# Autodesk Inventor assembly: ANDGATEASSEMBLY
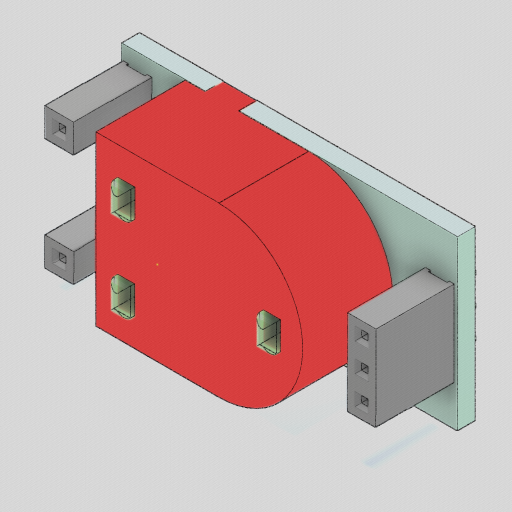
[picture p0: Inventor's stored thumbnail of the model, 512x512]
Saved by Autodesk Inventor 2024.3 (Build 283343000, 343)
## iProperties
Created: 2024-01-22
Part Number: ANDGATEASSEMBLY
Document SubType Name: Assembly
Designer: Jetsan
Author: Jetsan
## Documents named in this file (4)
- C:\Git\DigitalLogicProject\Models\ANDGATE\ANDGATEASSEMBLY.iam
- C:\Git\DigitalLogicProject\Models\LIGHTPIPING\LightPipe.ipt
- C:\Git\DigitalLogicProject\PCBS\GATE\GATE PCB.ipt
- C:\Git\DigitalLogicProject\Models\ANDGATE\ANDGATE.ipt
## Components (5 placed, 3 different names)
1. LightPipe:1 — Mate:3
2. LightPipe:2 — Mate:4
3. ANDGATE:1
4. GATE PCB:1 — Mate:3, Mate:4, Mate:10
5. LightPipe:3 — Mate:10
## Relationships (11: Mate 10, Flush 1)
- Mate:3: LightPipe:1 ↔ GATE PCB:1
- Mate:4: LightPipe:2 ↔ GATE PCB:1
- [Flush]: ANDGATE:1 ↔ GATE PCB:1
- [Mate]: ANDGATE:1 ↔ GATE PCB:1
- [Mate]: LightPipe:1 ↔ ANDGATE:1
- [Mate]: LightPipe:1 ↔ ANDGATE:1
- [Mate]: LightPipe:2 ↔ ANDGATE:1
- [Mate]: LightPipe:2 ↔ ANDGATE:1
- Mate:10: GATE PCB:1 ↔ LightPipe:3
- [Mate]: ANDGATE:1 ↔ LightPipe:3
- [Mate]: ANDGATE:1 ↔ LightPipe:3
